# Autodesk Inventor assembly: 底座
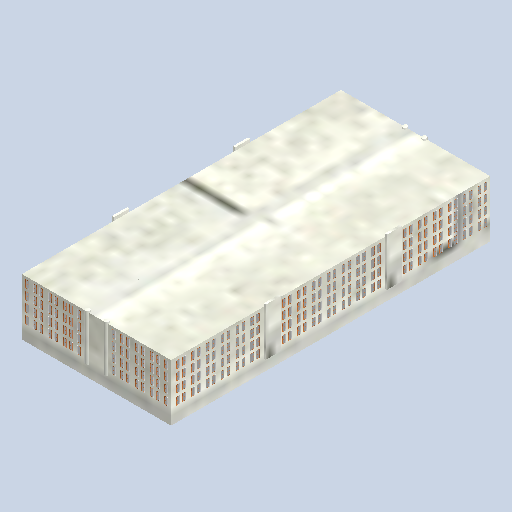
[picture p0: Inventor's stored thumbnail of the model, 512x512]
Saved by Autodesk Inventor 2024.2 (Build 282272000, 272)
## iProperties
Created: 2024-06-05
Part Number: 底座
Document SubType Name: Assembly
Designer: User
Author: User
## Documents named in this file (3)
- C:\Users\User\OneDrive - 國立中山大學\桌面\創客基礎\final_project\底座\底座.iam
- C:\Users\User\OneDrive - 國立中山大學\桌面\創客基礎\final_project\底座\底部.ipt
- C:\Users\User\OneDrive - 國立中山大學\桌面\創客基礎\final_project\組合窗_無底.iam
## Components (433 placed, 2 different names)
1. 底部:1 — 貼合:1, 貼合:2, 齊平:1, 貼合:3, 貼合:4, 齊平:2, 貼合:5, 貼合:6, 齊平:3, 貼合:7, 貼合:8, 齊平:4, 貼合:9, 貼合:10, 齊平:5, 貼合:11, 貼合:12, 貼合:13, 齊平:6, 貼合:14, 貼合:15, 齊平:7, 貼合:16, 貼合:17, 齊平:8
2. 組合窗_無底:54 [sub-assembly] — 貼合:9, 貼合:10, 齊平:5
3. 組合窗_無底:55 [sub-assembly]
4. 組合窗_無底:56 [sub-assembly]
5. 組合窗_無底:57 [sub-assembly]
6. 組合窗_無底:58 [sub-assembly]
7. 組合窗_無底:59 [sub-assembly]
8. 組合窗_無底:60 [sub-assembly]
9. 組合窗_無底:61 [sub-assembly]
10. 組合窗_無底:62 [sub-assembly]
11. 組合窗_無底:63 [sub-assembly]
12. 組合窗_無底:64 [sub-assembly]
13. 組合窗_無底:65 [sub-assembly]
14. 組合窗_無底:66 [sub-assembly]
15. 組合窗_無底:67 [sub-assembly]
16. 組合窗_無底:68 [sub-assembly]
17. 組合窗_無底:69 [sub-assembly]
18. 組合窗_無底:70 [sub-assembly]
19. 組合窗_無底:71 [sub-assembly]
20. 組合窗_無底:72 [sub-assembly]
21. 組合窗_無底:73 [sub-assembly]
22. 組合窗_無底:74 [sub-assembly]
23. 組合窗_無底:75 [sub-assembly]
24. 組合窗_無底:76 [sub-assembly]
25. 組合窗_無底:77 [sub-assembly]
26. 組合窗_無底:78 [sub-assembly]
27. 組合窗_無底:79 [sub-assembly]
28. 組合窗_無底:80 [sub-assembly]
29. 組合窗_無底:81 [sub-assembly]
30. 組合窗_無底:82 [sub-assembly]
31. 組合窗_無底:83 [sub-assembly]
32. 組合窗_無底:84 [sub-assembly]
33. 組合窗_無底:85 [sub-assembly]
34. 組合窗_無底:86 [sub-assembly]
35. 組合窗_無底:87 [sub-assembly]
36. 組合窗_無底:88 [sub-assembly]
37. 組合窗_無底:89 [sub-assembly]
38. 組合窗_無底:90 [sub-assembly]
39. 組合窗_無底:91 [sub-assembly]
40. 組合窗_無底:92 [sub-assembly]
41. 組合窗_無底:93 [sub-assembly]
42. 組合窗_無底:94 [sub-assembly]
43. 組合窗_無底:95 [sub-assembly]
44. 組合窗_無底:96 [sub-assembly]
45. 組合窗_無底:97 [sub-assembly]
46. 組合窗_無底:98 [sub-assembly]
47. 組合窗_無底:99 [sub-assembly]
48. 組合窗_無底:100 [sub-assembly]
49. 組合窗_無底:101 [sub-assembly]
50. 組合窗_無底:102 [sub-assembly]
51. 組合窗_無底:103 [sub-assembly]
52. 組合窗_無底:104 [sub-assembly]
53. 組合窗_無底:105 [sub-assembly]
54. 組合窗_無底:106 [sub-assembly]
55. 組合窗_無底:107 [sub-assembly]
56. 組合窗_無底:108 [sub-assembly]
57. 組合窗_無底:109 [sub-assembly]
58. 組合窗_無底:3 [sub-assembly] — 貼合:7, 貼合:8, 齊平:4, 貼合:11
59. 組合窗_無底:110 [sub-assembly]
60. 組合窗_無底:111 [sub-assembly]
61. 組合窗_無底:112 [sub-assembly]
62. 組合窗_無底:113 [sub-assembly]
63. 組合窗_無底:114 [sub-assembly]
64. 組合窗_無底:115 [sub-assembly]
65. 組合窗_無底:116 [sub-assembly]
66. 組合窗_無底:165 [sub-assembly]
67. 組合窗_無底:166 [sub-assembly]
68. 組合窗_無底:167 [sub-assembly]
69. 組合窗_無底:168 [sub-assembly]
70. 組合窗_無底:169 [sub-assembly]
71. 組合窗_無底:170 [sub-assembly]
72. 組合窗_無底:171 [sub-assembly]
73. 組合窗_無底:172 [sub-assembly]
74. 組合窗_無底:6 [sub-assembly] — 貼合:3, 貼合:4, 齊平:2
75. 組合窗_無底:221 [sub-assembly]
76. 組合窗_無底:318 [sub-assembly]
77. 組合窗_無底:415 [sub-assembly]
78. 組合窗_無底:512 [sub-assembly]
79. 組合窗_無底:609 [sub-assembly]
80. 組合窗_無底:706 [sub-assembly]
81. 組合窗_無底:803 [sub-assembly]
82. 組合窗_無底:852 [sub-assembly]
83. 組合窗_無底:853 [sub-assembly]
84. 組合窗_無底:854 [sub-assembly]
85. 組合窗_無底:855 [sub-assembly]
86. 組合窗_無底:856 [sub-assembly]
87. 組合窗_無底:857 [sub-assembly]
88. 組合窗_無底:858 [sub-assembly]
89. 組合窗_無底:859 [sub-assembly]
90. 組合窗_無底:955 [sub-assembly] — 貼合:16, 貼合:17, 齊平:8
91. 組合窗_無底:956 [sub-assembly]
92. 組合窗_無底:957 [sub-assembly]
93. 組合窗_無底:958 [sub-assembly]
94. 組合窗_無底:959 [sub-assembly]
95. 組合窗_無底:960 [sub-assembly]
96. 組合窗_無底:961 [sub-assembly]
97. 組合窗_無底:962 [sub-assembly]
98. 組合窗_無底:963 [sub-assembly]
99. 組合窗_無底:964 [sub-assembly]
100. 組合窗_無底:965 [sub-assembly]
101. 組合窗_無底:966 [sub-assembly]
102. 組合窗_無底:967 [sub-assembly]
103. 組合窗_無底:968 [sub-assembly]
104. 組合窗_無底:969 [sub-assembly]
105. 組合窗_無底:970 [sub-assembly]
106. 組合窗_無底:971 [sub-assembly]
107. 組合窗_無底:972 [sub-assembly]
108. 組合窗_無底:973 [sub-assembly]
109. 組合窗_無底:974 [sub-assembly]
110. 組合窗_無底:975 [sub-assembly]
111. 組合窗_無底:976 [sub-assembly]
112. 組合窗_無底:977 [sub-assembly]
113. 組合窗_無底:978 [sub-assembly]
114. 組合窗_無底:979 [sub-assembly]
115. 組合窗_無底:980 [sub-assembly]
116. 組合窗_無底:981 [sub-assembly]
117. 組合窗_無底:982 [sub-assembly]
118. 組合窗_無底:983 [sub-assembly]
119. 組合窗_無底:984 [sub-assembly]
120. 組合窗_無底:985 [sub-assembly]
121. 組合窗_無底:986 [sub-assembly]
122. 組合窗_無底:987 [sub-assembly]
123. 組合窗_無底:988 [sub-assembly]
124. 組合窗_無底:989 [sub-assembly]
125. 組合窗_無底:990 [sub-assembly]
126. 組合窗_無底:991 [sub-assembly]
127. 組合窗_無底:992 [sub-assembly]
128. 組合窗_無底:993 [sub-assembly]
129. 組合窗_無底:994 [sub-assembly]
130. 組合窗_無底:995 [sub-assembly]
131. 組合窗_無底:996 [sub-assembly]
132. 組合窗_無底:997 [sub-assembly]
133. 組合窗_無底:998 [sub-assembly]
134. 組合窗_無底:999 [sub-assembly]
135. 組合窗_無底:1000 [sub-assembly]
136. 組合窗_無底:1001 [sub-assembly]
137. 組合窗_無底:1002 [sub-assembly]
138. 組合窗_無底:1003 [sub-assembly]
139. 組合窗_無底:1004 [sub-assembly]
140. 組合窗_無底:1005 [sub-assembly]
141. 組合窗_無底:1006 [sub-assembly]
142. 組合窗_無底:1007 [sub-assembly]
143. 組合窗_無底:1008 [sub-assembly]
144. 組合窗_無底:1009 [sub-assembly]
145. 組合窗_無底:1010 [sub-assembly]
146. 組合窗_無底:117 [sub-assembly] — 貼合:12, 貼合:13, 齊平:6
147. 組合窗_無底:118 [sub-assembly]
148. 組合窗_無底:119 [sub-assembly]
149. 組合窗_無底:120 [sub-assembly]
150. 組合窗_無底:121 [sub-assembly]
151. 組合窗_無底:122 [sub-assembly]
152. 組合窗_無底:123 [sub-assembly]
153. 組合窗_無底:124 [sub-assembly]
154. 組合窗_無底:125 [sub-assembly]
155. 組合窗_無底:126 [sub-assembly]
156. 組合窗_無底:127 [sub-assembly]
157. 組合窗_無底:128 [sub-assembly]
158. 組合窗_無底:129 [sub-assembly]
159. 組合窗_無底:130 [sub-assembly]
160. 組合窗_無底:131 [sub-assembly]
161. 組合窗_無底:132 [sub-assembly]
162. 組合窗_無底:133 [sub-assembly]
163. 組合窗_無底:134 [sub-assembly]
164. 組合窗_無底:135 [sub-assembly]
165. 組合窗_無底:136 [sub-assembly]
166. 組合窗_無底:137 [sub-assembly]
167. 組合窗_無底:138 [sub-assembly]
168. 組合窗_無底:139 [sub-assembly]
169. 組合窗_無底:140 [sub-assembly]
170. 組合窗_無底:141 [sub-assembly]
171. 組合窗_無底:142 [sub-assembly]
172. 組合窗_無底:143 [sub-assembly]
173. 組合窗_無底:144 [sub-assembly]
174. 組合窗_無底:145 [sub-assembly]
175. 組合窗_無底:146 [sub-assembly]
176. 組合窗_無底:147 [sub-assembly]
177. 組合窗_無底:148 [sub-assembly]
178. 組合窗_無底:149 [sub-assembly]
179. 組合窗_無底:150 [sub-assembly]
180. 組合窗_無底:151 [sub-assembly]
181. 組合窗_無底:152 [sub-assembly]
182. 組合窗_無底:153 [sub-assembly]
183. 組合窗_無底:154 [sub-assembly]
184. 組合窗_無底:155 [sub-assembly]
185. 組合窗_無底:156 [sub-assembly]
186. 組合窗_無底:157 [sub-assembly]
187. 組合窗_無底:158 [sub-assembly]
188. 組合窗_無底:159 [sub-assembly]
189. 組合窗_無底:160 [sub-assembly]
190. 組合窗_無底:161 [sub-assembly]
191. 組合窗_無底:162 [sub-assembly]
192. 組合窗_無底:163 [sub-assembly]
193. 組合窗_無底:164 [sub-assembly]
194. 組合窗_無底:804 [sub-assembly] — 貼合:14, 貼合:15, 齊平:7
195. 組合窗_無底:805 [sub-assembly]
196. 組合窗_無底:806 [sub-assembly]
197. 組合窗_無底:807 [sub-assembly]
198. 組合窗_無底:808 [sub-assembly]
199. 組合窗_無底:809 [sub-assembly]
200. 組合窗_無底:810 [sub-assembly]
201. 組合窗_無底:811 [sub-assembly]
202. 組合窗_無底:812 [sub-assembly]
203. 組合窗_無底:813 [sub-assembly]
204. 組合窗_無底:814 [sub-assembly]
205. 組合窗_無底:815 [sub-assembly]
206. 組合窗_無底:816 [sub-assembly]
207. 組合窗_無底:817 [sub-assembly]
208. 組合窗_無底:818 [sub-assembly]
209. 組合窗_無底:819 [sub-assembly]
210. 組合窗_無底:820 [sub-assembly]
211. 組合窗_無底:821 [sub-assembly]
212. 組合窗_無底:822 [sub-assembly]
213. 組合窗_無底:823 [sub-assembly]
214. 組合窗_無底:824 [sub-assembly]
215. 組合窗_無底:825 [sub-assembly]
216. 組合窗_無底:826 [sub-assembly]
217. 組合窗_無底:827 [sub-assembly]
218. 組合窗_無底:828 [sub-assembly]
219. 組合窗_無底:829 [sub-assembly]
220. 組合窗_無底:830 [sub-assembly]
221. 組合窗_無底:831 [sub-assembly]
222. 組合窗_無底:832 [sub-assembly]
223. 組合窗_無底:833 [sub-assembly]
224. 組合窗_無底:834 [sub-assembly]
225. 組合窗_無底:835 [sub-assembly]
226. 組合窗_無底:836 [sub-assembly]
227. 組合窗_無底:837 [sub-assembly]
228. 組合窗_無底:838 [sub-assembly]
229. 組合窗_無底:839 [sub-assembly]
230. 組合窗_無底:840 [sub-assembly]
231. 組合窗_無底:841 [sub-assembly]
232. 組合窗_無底:842 [sub-assembly]
233. 組合窗_無底:843 [sub-assembly]
234. 組合窗_無底:844 [sub-assembly]
235. 組合窗_無底:845 [sub-assembly]
236. 組合窗_無底:846 [sub-assembly]
237. 組合窗_無底:847 [sub-assembly]
238. 組合窗_無底:848 [sub-assembly]
239. 組合窗_無底:849 [sub-assembly]
240. 組合窗_無底:850 [sub-assembly]
241. 組合窗_無底:851 [sub-assembly]
242. 組合窗_無底:1 [sub-assembly] — 貼合:1, 貼合:2, 齊平:1
243. 組合窗_無底:860 [sub-assembly]
244. 組合窗_無底:861 [sub-assembly]
245. 組合窗_無底:862 [sub-assembly]
246. 組合窗_無底:863 [sub-assembly]
247. 組合窗_無底:864 [sub-assembly]
248. 組合窗_無底:865 [sub-assembly]
249. 組合窗_無底:866 [sub-assembly]
250. 組合窗_無底:867 [sub-assembly]
251. 組合窗_無底:868 [sub-assembly]
252. 組合窗_無底:869 [sub-assembly]
253. 組合窗_無底:870 [sub-assembly]
254. 組合窗_無底:871 [sub-assembly]
255. 組合窗_無底:872 [sub-assembly]
256. 組合窗_無底:873 [sub-assembly]
257. 組合窗_無底:874 [sub-assembly]
258. 組合窗_無底:875 [sub-assembly]
259. 組合窗_無底:876 [sub-assembly]
260. 組合窗_無底:877 [sub-assembly]
261. 組合窗_無底:878 [sub-assembly]
262. 組合窗_無底:879 [sub-assembly]
263. 組合窗_無底:880 [sub-assembly]
264. 組合窗_無底:881 [sub-assembly]
265. 組合窗_無底:882 [sub-assembly]
266. 組合窗_無底:883 [sub-assembly]
267. 組合窗_無底:884 [sub-assembly]
268. 組合窗_無底:885 [sub-assembly]
269. 組合窗_無底:886 [sub-assembly]
270. 組合窗_無底:887 [sub-assembly]
271. 組合窗_無底:888 [sub-assembly]
272. 組合窗_無底:889 [sub-assembly]
273. 組合窗_無底:890 [sub-assembly]
274. 組合窗_無底:891 [sub-assembly]
275. 組合窗_無底:892 [sub-assembly]
276. 組合窗_無底:893 [sub-assembly]
277. 組合窗_無底:894 [sub-assembly]
278. 組合窗_無底:895 [sub-assembly]
279. 組合窗_無底:896 [sub-assembly]
280. 組合窗_無底:897 [sub-assembly]
281. 組合窗_無底:898 [sub-assembly]
282. 組合窗_無底:899 [sub-assembly]
283. 組合窗_無底:900 [sub-assembly]
284. 組合窗_無底:901 [sub-assembly]
285. 組合窗_無底:902 [sub-assembly]
286. 組合窗_無底:903 [sub-assembly]
287. 組合窗_無底:904 [sub-assembly]
288. 組合窗_無底:905 [sub-assembly]
289. 組合窗_無底:906 [sub-assembly]
290. 組合窗_無底:907 [sub-assembly]
291. 組合窗_無底:908 [sub-assembly]
292. 組合窗_無底:909 [sub-assembly]
293. 組合窗_無底:910 [sub-assembly]
294. 組合窗_無底:911 [sub-assembly]
295. 組合窗_無底:912 [sub-assembly]
296. 組合窗_無底:913 [sub-assembly]
297. 組合窗_無底:914 [sub-assembly]
298. 組合窗_無底:915 [sub-assembly]
299. 組合窗_無底:916 [sub-assembly]
300. 組合窗_無底:917 [sub-assembly]
301. 組合窗_無底:918 [sub-assembly]
302. 組合窗_無底:919 [sub-assembly]
303. 組合窗_無底:920 [sub-assembly]
304. 組合窗_無底:921 [sub-assembly]
305. 組合窗_無底:922 [sub-assembly]
306. 組合窗_無底:923 [sub-assembly]
307. 組合窗_無底:924 [sub-assembly]
308. 組合窗_無底:925 [sub-assembly]
309. 組合窗_無底:926 [sub-assembly]
310. 組合窗_無底:927 [sub-assembly]
311. 組合窗_無底:928 [sub-assembly]
312. 組合窗_無底:929 [sub-assembly]
313. 組合窗_無底:930 [sub-assembly]
314. 組合窗_無底:931 [sub-assembly]
315. 組合窗_無底:932 [sub-assembly]
316. 組合窗_無底:933 [sub-assembly]
317. 組合窗_無底:934 [sub-assembly]
318. 組合窗_無底:935 [sub-assembly]
319. 組合窗_無底:936 [sub-assembly]
320. 組合窗_無底:937 [sub-assembly]
321. 組合窗_無底:938 [sub-assembly]
322. 組合窗_無底:939 [sub-assembly]
323. 組合窗_無底:940 [sub-assembly]
324. 組合窗_無底:941 [sub-assembly]
325. 組合窗_無底:942 [sub-assembly]
326. 組合窗_無底:943 [sub-assembly]
327. 組合窗_無底:944 [sub-assembly]
328. 組合窗_無底:945 [sub-assembly]
329. 組合窗_無底:946 [sub-assembly]
330. 組合窗_無底:947 [sub-assembly]
331. 組合窗_無底:948 [sub-assembly]
332. 組合窗_無底:949 [sub-assembly]
333. 組合窗_無底:950 [sub-assembly]
334. 組合窗_無底:951 [sub-assembly]
335. 組合窗_無底:952 [sub-assembly]
336. 組合窗_無底:953 [sub-assembly]
337. 組合窗_無底:954 [sub-assembly]
338. 組合窗_無底:4 [sub-assembly] — 貼合:5, 貼合:6, 齊平:3
339. 組合窗_無底:7 [sub-assembly]
340. 組合窗_無底:8 [sub-assembly]
341. 組合窗_無底:9 [sub-assembly]
342. 組合窗_無底:10 [sub-assembly]
343. 組合窗_無底:11 [sub-assembly]
344. 組合窗_無底:12 [sub-assembly]
345. 組合窗_無底:13 [sub-assembly]
346. 組合窗_無底:14 [sub-assembly]
347. 組合窗_無底:15 [sub-assembly]
348. 組合窗_無底:16 [sub-assembly]
349. 組合窗_無底:17 [sub-assembly]
350. 組合窗_無底:18 [sub-assembly]
351. 組合窗_無底:19 [sub-assembly]
352. 組合窗_無底:20 [sub-assembly]
353. 組合窗_無底:21 [sub-assembly]
354. 組合窗_無底:22 [sub-assembly]
355. 組合窗_無底:23 [sub-assembly]
356. 組合窗_無底:24 [sub-assembly]
357. 組合窗_無底:25 [sub-assembly]
358. 組合窗_無底:26 [sub-assembly]
359. 組合窗_無底:27 [sub-assembly]
360. 組合窗_無底:28 [sub-assembly]
361. 組合窗_無底:29 [sub-assembly]
362. 組合窗_無底:30 [sub-assembly]
363. 組合窗_無底:31 [sub-assembly]
364. 組合窗_無底:32 [sub-assembly]
365. 組合窗_無底:33 [sub-assembly]
366. 組合窗_無底:34 [sub-assembly]
367. 組合窗_無底:35 [sub-assembly]
368. 組合窗_無底:36 [sub-assembly]
369. 組合窗_無底:37 [sub-assembly]
370. 組合窗_無底:38 [sub-assembly]
371. 組合窗_無底:39 [sub-assembly]
372. 組合窗_無底:40 [sub-assembly]
373. 組合窗_無底:41 [sub-assembly]
374. 組合窗_無底:42 [sub-assembly]
375. 組合窗_無底:43 [sub-assembly]
376. 組合窗_無底:44 [sub-assembly]
377. 組合窗_無底:45 [sub-assembly]
378. 組合窗_無底:46 [sub-assembly]
379. 組合窗_無底:47 [sub-assembly]
380. 組合窗_無底:48 [sub-assembly]
381. 組合窗_無底:49 [sub-assembly]
382. 組合窗_無底:50 [sub-assembly]
383. 組合窗_無底:51 [sub-assembly]
384. 組合窗_無底:52 [sub-assembly]
385. 組合窗_無底:53 [sub-assembly]
386. 組合窗_無底:173 [sub-assembly]
387. 組合窗_無底:174 [sub-assembly]
388. 組合窗_無底:175 [sub-assembly]
389. 組合窗_無底:176 [sub-assembly]
390. 組合窗_無底:177 [sub-assembly]
391. 組合窗_無底:178 [sub-assembly]
392. 組合窗_無底:179 [sub-assembly]
393. 組合窗_無底:180 [sub-assembly]
394. 組合窗_無底:181 [sub-assembly]
395. 組合窗_無底:182 [sub-assembly]
396. 組合窗_無底:183 [sub-assembly]
397. 組合窗_無底:184 [sub-assembly]
398. 組合窗_無底:185 [sub-assembly]
399. 組合窗_無底:186 [sub-assembly]
400. 組合窗_無底:187 [sub-assembly]
401. 組合窗_無底:188 [sub-assembly]
402. 組合窗_無底:189 [sub-assembly]
403. 組合窗_無底:190 [sub-assembly]
404. 組合窗_無底:191 [sub-assembly]
405. 組合窗_無底:192 [sub-assembly]
406. 組合窗_無底:193 [sub-assembly]
407. 組合窗_無底:194 [sub-assembly]
408. 組合窗_無底:195 [sub-assembly]
409. 組合窗_無底:196 [sub-assembly]
410. 組合窗_無底:197 [sub-assembly]
411. 組合窗_無底:198 [sub-assembly]
412. 組合窗_無底:199 [sub-assembly]
413. 組合窗_無底:200 [sub-assembly]
414. 組合窗_無底:201 [sub-assembly]
415. 組合窗_無底:202 [sub-assembly]
416. 組合窗_無底:203 [sub-assembly]
417. 組合窗_無底:204 [sub-assembly]
418. 組合窗_無底:205 [sub-assembly]
419. 組合窗_無底:206 [sub-assembly]
420. 組合窗_無底:207 [sub-assembly]
421. 組合窗_無底:208 [sub-assembly]
422. 組合窗_無底:209 [sub-assembly]
423. 組合窗_無底:210 [sub-assembly]
424. 組合窗_無底:211 [sub-assembly]
425. 組合窗_無底:212 [sub-assembly]
426. 組合窗_無底:213 [sub-assembly]
427. 組合窗_無底:214 [sub-assembly]
428. 組合窗_無底:215 [sub-assembly]
429. 組合窗_無底:216 [sub-assembly]
430. 組合窗_無底:217 [sub-assembly]
431. 組合窗_無底:218 [sub-assembly]
432. 組合窗_無底:219 [sub-assembly]
433. 組合窗_無底:220 [sub-assembly]
## Component patterns: (7 elements), (2 elements), (2 elements), (2 elements), (2 elements), (7 elements), (8 elements, first: 組合窗_無底:54), 元件陣列 4:2 (8 elements), 元件陣列 4:3 (8 elements), 元件陣列 4:4 (8 elements), 元件陣列 4:5 (8 elements), 元件陣列 4:6 (8 elements), 元件陣列 4:7 (8 elements), (3 elements), (8 elements, first: 組合窗_無底:3), 元件陣列 8:2 (3 elements), 元件陣列 6:2 (8 elements), (6 elements), 元件陣列 3:2 (6 elements), (3 elements), (8 elements, first: 組合窗_無底:6), 元件陣列 13:2 (3 elements), 元件陣列 11:2 (8 elements), (6 elements), 元件陣列 16:2 (6 elements), (8 elements, first: 組合窗_無底:955), 元件陣列 18:2 (8 elements), 元件陣列 18:3 (8 elements), 元件陣列 18:4 (8 elements), 元件陣列 18:5 (8 elements), 元件陣列 18:6 (8 elements), 元件陣列 18:7 (8 elements), (8 elements, first: 組合窗_無底:117), 元件陣列 7:2 (8 elements), 元件陣列 7:3 (8 elements), 元件陣列 7:4 (8 elements), 元件陣列 7:5 (8 elements), 元件陣列 7:6 (8 elements), (2 elements), 元件陣列 2:2 (2 elements), 元件陣列 2:3 (2 elements), 元件陣列 2:4 (2 elements), 元件陣列 2:5 (2 elements), 元件陣列 2:6 (2 elements), 元件陣列 2:7 (2 elements), 元件陣列 2:8 (2 elements), 元件陣列 2:9 (2 elements), 元件陣列 2:10 (2 elements), 元件陣列 2:11 (2 elements), 元件陣列 2:12 (2 elements), (8 elements, first: 組合窗_無底:804), 元件陣列 12:2 (8 elements), 元件陣列 12:3 (8 elements), 元件陣列 12:4 (8 elements), 元件陣列 12:5 (8 elements), 元件陣列 12:6 (8 elements), (8 elements, first: 組合窗_無底:1), 元件陣列 15:2 (8 elements), 元件陣列 15:3 (8 elements), 元件陣列 15:4 (8 elements), 元件陣列 15:5 (8 elements), 元件陣列 15:6 (8 elements), 元件陣列 15:7 (8 elements), 元件陣列 15:8 (8 elements), 元件陣列 15:9 (8 elements), 元件陣列 15:10 (8 elements), 元件陣列 15:11 (8 elements), 元件陣列 15:12 (8 elements), (4 elements, first: 組合窗_無底:4), 元件陣列 1:2 (4 elements), 元件陣列 1:3 (4 elements), 元件陣列 1:4 (4 elements), 元件陣列 1:5 (4 elements), 元件陣列 1:6 (4 elements), 元件陣列 1:7 (4 elements), 元件陣列 1:8 (4 elements), 元件陣列 1:9 (4 elements), 元件陣列 1:10 (4 elements), 元件陣列 1:11 (4 elements), 元件陣列 1:12 (4 elements), 元件陣列 1:13 (4 elements), 元件陣列 1:14 (4 elements), 元件陣列 1:15 (4 elements), 元件陣列 1:16 (4 elements), 元件陣列 1:17 (4 elements), 元件陣列 1:18 (4 elements), 元件陣列 1:19 (4 elements), 元件陣列 1:20 (4 elements), 元件陣列 1:21 (4 elements), 元件陣列 1:22 (4 elements), 元件陣列 1:23 (4 elements), 元件陣列 1:24 (4 elements)
## Relationships (25: Mate 17, Flush 8)
- 貼合:1 [Mate]: 底部:1 ↔ 組合窗_無底:1
- 貼合:2 [Mate]: 底部:1 ↔ 組合窗_無底:1
- 齊平:1 [Flush]: 底部:1 ↔ 組合窗_無底:1
- 貼合:3 [Mate]: 底部:1 ↔ 組合窗_無底:6
- 貼合:4 [Mate]: 底部:1 ↔ 組合窗_無底:6
- 齊平:2 [Flush]: 底部:1 ↔ 組合窗_無底:6
- 貼合:5 [Mate]: 底部:1 ↔ 組合窗_無底:4
- 貼合:6 [Mate]: 底部:1 ↔ 組合窗_無底:4
- 齊平:3 [Flush]: 底部:1 ↔ 組合窗_無底:4
- 貼合:7 [Mate]: 底部:1 ↔ 組合窗_無底:3
- 貼合:8 [Mate]: 底部:1 ↔ 組合窗_無底:3
- 齊平:4 [Flush]: 底部:1 ↔ 組合窗_無底:3
- 貼合:9 [Mate]: 底部:1 ↔ 組合窗_無底:54
- 貼合:10 [Mate]: 底部:1 ↔ 組合窗_無底:54
- 齊平:5 [Flush]: 底部:1 ↔ 組合窗_無底:54
- 貼合:11 [Mate]: 底部:1 ↔ 組合窗_無底:3
- 貼合:12 [Mate]: 底部:1 ↔ 組合窗_無底:117
- 貼合:13 [Mate]: 底部:1 ↔ 組合窗_無底:117
- 齊平:6 [Flush]: 底部:1 ↔ 組合窗_無底:117
- 貼合:14 [Mate]: 底部:1 ↔ 組合窗_無底:804
- 貼合:15 [Mate]: 底部:1 ↔ 組合窗_無底:804
- 齊平:7 [Flush]: 底部:1 ↔ 組合窗_無底:804
- 貼合:16 [Mate]: 底部:1 ↔ 組合窗_無底:955
- 貼合:17 [Mate]: 底部:1 ↔ 組合窗_無底:955
- 齊平:8 [Flush]: 底部:1 ↔ 組合窗_無底:955
